# Autodesk Inventor assembly: Ensemble_Relier_suspension
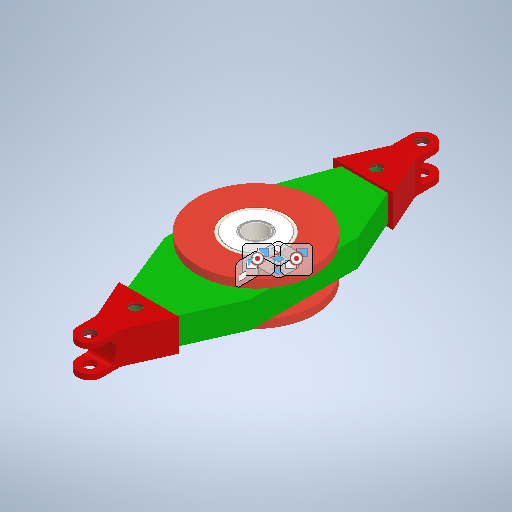
[picture p0: Inventor's stored thumbnail of the model, 512x512]
Saved by Autodesk Inventor 2026.2 (Build 302298010, 298A)
## iProperties
Created: 2026-03-16
Part Number: Ensemble_Relier_suspension
Document SubType Name: Assembly
Designer: genon
Author: genon
## Documents named in this file (5)
- C:\Users\genon\Documents\Henallux Passerelle\Projet de conception\Cassini T-X\Inventor\Suspension\Ensemble_Relier_suspension.iam
- C:\Users\genon\Documents\Henallux Passerelle\Projet de conception\Cassini T-X\Inventor\Suspension\Axe centrale.ipt
- C:\Users\genon\Documents\Henallux Passerelle\Projet de conception\Cassini T-X\Inventor\Suspension\Fixation_rotule_axe_centrale.ipt
- C:\Users\genon\Documents\Henallux Passerelle\Projet de conception\Cassini T-X\Inventor\Suspension\Rolling v2.ipt
- C:\Users\genon\Documents\Henallux Passerelle\Projet de conception\Cassini T-X\Inventor\Suspension\Axe centrale V2.ipt
## Components (7 placed, 4 different names)
1. Axe centrale:1 — Placage:7, Placage:8, Placage:9, Placage:10, Placage:11, Placage:12, Placage:17, Placage:18, Placage:19, Placage:20, Placage:21, Placage:22
2. Fixation_rotule_axe_centrale:1 — Placage:20, Placage:21, Placage:22
3. Fixation_rotule_axe_centrale:2 — Placage:17, Placage:18, Placage:19
4. Rolling v2:1 — Placage:15, Placage:16
5. Rolling v2:2 — Placage:13, Placage:14
6. Axe centrale V2:1 — Placage:7, Placage:8, Placage:9, Placage:15, Placage:16
7. Axe centrale V2:2 — Placage:10, Placage:11, Placage:12, Placage:13, Placage:14
## Relationships (16: Mate 16)
- Placage:7 [Mate]: Axe centrale:1 ↔ Axe centrale V2:1
- Placage:8 [Mate]: Axe centrale:1 ↔ Axe centrale V2:1
- Placage:9 [Mate]: Axe centrale:1 ↔ Axe centrale V2:1
- Placage:10 [Mate]: Axe centrale:1 ↔ Axe centrale V2:2
- Placage:11 [Mate]: Axe centrale:1 ↔ Axe centrale V2:2
- Placage:12 [Mate]: Axe centrale:1 ↔ Axe centrale V2:2
- Placage:13 [Mate]: Rolling v2:2 ↔ Axe centrale V2:2
- Placage:14 [Mate]: Rolling v2:2 ↔ Axe centrale V2:2
- Placage:15 [Mate]: Rolling v2:1 ↔ Axe centrale V2:1
- Placage:16 [Mate]: Rolling v2:1 ↔ Axe centrale V2:1
- Placage:17 [Mate]: Axe centrale:1 ↔ Fixation_rotule_axe_centrale:2
- Placage:18 [Mate]: Axe centrale:1 ↔ Fixation_rotule_axe_centrale:2
- Placage:19 [Mate]: Axe centrale:1 ↔ Fixation_rotule_axe_centrale:2
- Placage:20 [Mate]: Axe centrale:1 ↔ Fixation_rotule_axe_centrale:1
- Placage:21 [Mate]: Axe centrale:1 ↔ Fixation_rotule_axe_centrale:1
- Placage:22 [Mate]: Axe centrale:1 ↔ Fixation_rotule_axe_centrale:1
